# Autodesk Inventor assembly: PowerDetector
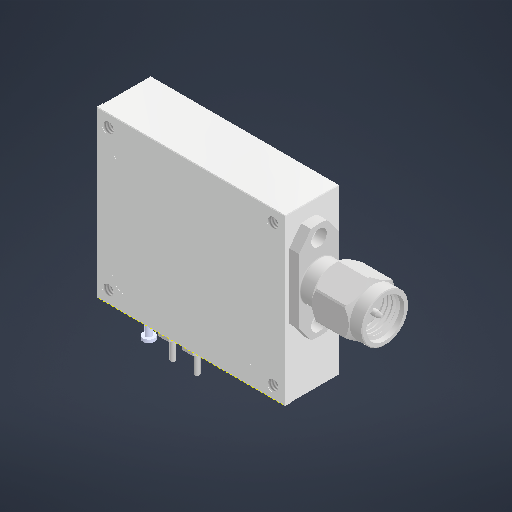
[picture p0: Inventor's stored thumbnail of the model, 512x512]
Saved by Autodesk Inventor 2026.2 (Build 302298010, 298A)
## iProperties
Created: 2026-06-22
Part Number: PowerDetector
Document SubType Name: Assembly
Designer: sonata
Author: sonata
## Documents named in this file (6)
- Z:\crush\mechanical\PAM-modules-mount\PowerDetector.iam
- Z:\crush\Front-Page\Analog-Signal-Components\PAX\PAM-2025\PAM-modules\detector-module\detector-module-v2\enclosure\Detector Box ND20.ipt
- Z:\crush\Front-Page\Analog-Signal-Components\PAX\PAM-2025\PAM-modules\detector-module\detector-module-v2\enclosure\Detector Lid ND20.ipt
- Z:\crush\mechanical\PAM-modules-mount\PE44032_3D\PE44032_3D\PE44032_3D.ipt
- Z:\crush\mechanical\PAM-modules-mount\1595-2\1595-2\1595-2.ipt
- Z:\crush\mechanical\PAM-modules-mount\FeedThroughCap.ipt
## Components (6 placed, 5 different names)
1. Detector Box ND20:1 — Mate:1, Mate:2, Mate:3, Mate:4, Mate:5, Mate:6, Mate:7, Mate:8
2. Detector Lid ND20:1 — Mate:1, Mate:4, Flush:1
3. PE44032_3D:1 — Mate:2
4. 1595-2:1 — Mate:3, Flush:1
5. FeedThroughCap:1 — Mate:5, Mate:7
6. FeedThroughCap:2 — Mate:6, Mate:8
## Relationships (9: Mate 8, Flush 1)
- Mate:1: Detector Box ND20:1 ↔ Detector Lid ND20:1
- Mate:2: Detector Box ND20:1 ↔ PE44032_3D:1
- Mate:3: Detector Box ND20:1 ↔ 1595-2:1
- Mate:4: Detector Box ND20:1 ↔ Detector Lid ND20:1
- Flush:1 (1.4 mm): Detector Lid ND20:1 ↔ 1595-2:1
- Mate:5: Detector Box ND20:1 ↔ FeedThroughCap:1
- Mate:6: Detector Box ND20:1 ↔ FeedThroughCap:2
- Mate:7: Detector Box ND20:1 ↔ FeedThroughCap:1
- Mate:8: Detector Box ND20:1 ↔ FeedThroughCap:2
